# Autodesk Inventor assembly: FE-00014
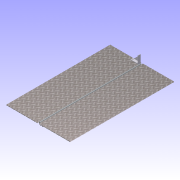
[picture p0: Inventor's stored thumbnail of the model, 180x180]
Saved by Autodesk Inventor 2012 (Build 160160000, 160)
## iProperties
Company: FIRST
Created: 2008-05-25
Part Number: FE-00014
Document SubType Name: Weldment
Designer: dfoster
Description: Field Entry Ramp
Weld Material: Welded Aluminum-6061
Title: Field Entry Ramp
Author: dfoster
## Documents named in this file (6)
- C:\Data Folder\FRC 2012 Field\Components\FE-00014.iam
- C:\Data Folder\FRC 2012 Field\Components\FE-00014-02.iam
- C:\Data Folder\FRC 2012 Field\Components\FE-00014-01.ipt
- C:\Data Folder\FRC 2012 Field\Components\FE-00014-03.ipt
- C:\Data Folder\FRC 2012 Field\Components\FE-00014-04.ipt
- C:\Data Folder\FRC 2012 Field\Components\FE-00014-05.ipt
## Components (6 placed, 5 different names)
1. FE-00014-02:1 [sub-assembly] — Mate:1, Tangent:1, Flush:1, Mate:2, Tangent:2, Flush:7
2. FE-00014-01:1 — Mate:1, Tangent:1, Flush:1, Flush:2, Mate:3, Flush:3, Flush:4
3. FE-00014-01:2 — Mate:2, Flush:2, Tangent:2, Flush:6
4. FE-00014-03:1 — Flush:6, Flush:7
5. FE-00014-04:1 — Mate:3, Flush:3, Flush:4, Mate:4, Flush:5, Mate:5
6. FE-00014-05:1 — Mate:4, Flush:5, Mate:5
## Relationships (15: Flush 7, Mate 6, Tangent 2)
- Mate:1: FE-00014-02:1 ↔ FE-00014-01:1
- Tangent:1 (0.7937 mm): FE-00014-02:1 ↔ FE-00014-01:1
- Flush:1 (-12.7 mm): FE-00014-02:1 ↔ FE-00014-01:1
- Mate:2: FE-00014-02:1 ↔ FE-00014-01:2
- Flush:2: FE-00014-01:1 ↔ FE-00014-01:2
- Tangent:2 (0.7937 mm): FE-00014-02:1 ↔ FE-00014-01:2
- Mate:3: FE-00014-01:1 ↔ FE-00014-04:1
- Flush:3: FE-00014-01:1 ↔ FE-00014-04:1
- Flush:4 (6.35 mm): FE-00014-01:1 ↔ FE-00014-04:1
- Mate:4: FE-00014-04:1 ↔ FE-00014-05:1
- Flush:5: FE-00014-04:1 ↔ FE-00014-05:1
- Mate:5: FE-00014-04:1 ↔ FE-00014-05:1
- [Mate]: FE-00014-02:1 ↔ FE-00014-03:1
- Flush:6: FE-00014-01:2 ↔ FE-00014-03:1
- Flush:7: FE-00014-02:1 ↔ FE-00014-03:1
